# Autodesk Inventor assembly: 1_Body
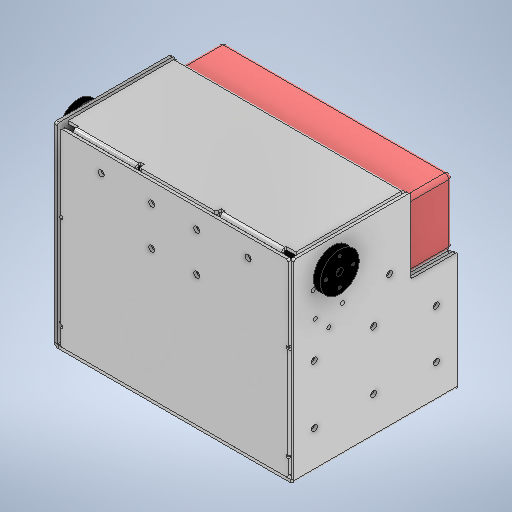
[picture p0: Inventor's stored thumbnail of the model, 512x512]
Saved by Autodesk Inventor 2025.2 (Build 292293000, 293)
## iProperties
Created: 2025-05-30
Part Number: 1_Body
Document SubType Name: Assembly
Designer: chris
Author: chris
## Documents named in this file (13)
- C:\Users\chris\Documents\Inventor\RHp_Humanoid_ver1\Assembly\1_Body.iam
- C:\Users\chris\Documents\Inventor\RHp_Humanoid_ver1\Part\Frame\Body\body_main_frame.ipt
- C:\Users\chris\Documents\Inventor\RHp_Humanoid_ver1\Part\Frame\Body\body_back_frame.ipt
- C:\Users\chris\Documents\Inventor\RHp_Humanoid_ver1\Part\Frame\Body\body_front_frame.ipt
- C:\Users\chris\Documents\Inventor\RHp_Humanoid_ver1\Part\Frame\Body\body_middle_frame.ipt
- C:\Users\chris\Documents\Inventor\RHp_Humanoid_ver1\Part\Frame\Body\body_motor_L_frame.ipt
- C:\Users\chris\Documents\Inventor\RHp_Humanoid_ver1\Part\Frame\Body\body_motor_R_frame.ipt
- C:\Users\chris\Documents\Inventor\RHp_Humanoid_ver1\Part\Frame\Body\body_top_frame.ipt
- C:\Users\chris\Documents\Inventor\RHp_Humanoid_ver1\Part\Other Parts\Servo_Driver.ipt
- C:\Users\chris\Documents\Inventor\RHp_Humanoid_ver1\Part\Other Parts\Battery_Pack.ipt
- C:\Users\chris\Documents\Inventor\RHp_Humanoid_ver1\Part\Other Parts\jetson_orin_super.ipt
- C:\Users\chris\Documents\Inventor\RHp_Humanoid_ver1\Part\HTD-45H, Horn\Horn\Top Horn.ipt
- C:\Users\chris\Documents\Inventor\RHp_Humanoid_ver1\Part\HTD-45H, Horn\HTD-45H\HTD-45H.iam
## Components (14 placed, 12 different names)
1. body_main_frame:1 — Mate:3, Flush:2, Mate:4, Mate:5, Flush:3, Flush:4, Mate:6, Flush:5, Mate:8, Mate:10, Mate:11, Flush:9, Flush:10, Mate:16, Mate:18, Flush:13, Mate:30, Flush:30, Flush:31, Mate:31, Mate:33
2. body_back_frame:1 — Mate:3, Flush:2, Mate:4, Mate:19
3. body_front_frame:1 — Mate:5, Flush:3, Flush:4, Flush:6, Mate:7, Flush:7, Mate:9, Flush:8
4. body_middle_frame:1 — Mate:6, Flush:5, Flush:6, Mate:17, Mate:28, Flush:29, Mate:29, Flush:32, Mate:32, Flush:33, Mate:34
5. body_motor_L_frame:1 — Mate:7, Flush:7, Mate:8
6. body_motor_R_frame:1 — Mate:9, Mate:10, Flush:8
7. body_top_frame:1 — Mate:11, Flush:9, Flush:10, Mate:20
8. Servo_Driver:1 — Mate:16, Mate:17, Mate:18
9. Battery_Pack:1 — Mate:19, Mate:20, Flush:13
10. jetson_orin_super:1 — Mate:28, Flush:29, Mate:29
11. Top Horn:1 — Rotational:1
12. Top Horn:2 — Rotational:2
13. HTD-45H:1 [sub-assembly] — Flush:32, Mate:31, Mate:32, Rotational:2
14. HTD-45H:2 [sub-assembly] — Flush:33, Mate:33, Mate:34, Rotational:1
## Relationships (38: Mate 21, Flush 15, RevoluteJoint 2)
- Mate:3: body_main_frame:1 ↔ body_back_frame:1
- Flush:2: body_main_frame:1 ↔ body_back_frame:1
- Mate:4: body_main_frame:1 ↔ body_back_frame:1
- Mate:5: body_main_frame:1 ↔ body_front_frame:1
- Flush:3 (1.5 mm): body_main_frame:1 ↔ body_front_frame:1
- Flush:4: body_main_frame:1 ↔ body_front_frame:1
- Mate:6: body_main_frame:1 ↔ body_middle_frame:1
- Flush:5 (1.5 mm): body_main_frame:1 ↔ body_middle_frame:1
- Flush:6 (-30 mm): body_front_frame:1 ↔ body_middle_frame:1
- Mate:7: body_front_frame:1 ↔ body_motor_L_frame:1
- Flush:7: body_front_frame:1 ↔ body_motor_L_frame:1
- Mate:8 (40 mm): body_main_frame:1 ↔ body_motor_L_frame:1
- Mate:9: body_front_frame:1 ↔ body_motor_R_frame:1
- Mate:10 (40 mm): body_main_frame:1 ↔ body_motor_R_frame:1
- Mate:11: body_main_frame:1 ↔ body_top_frame:1
- Flush:8: body_front_frame:1 ↔ body_motor_R_frame:1
- Flush:9: body_main_frame:1 ↔ body_top_frame:1
- Flush:10 (1.5 mm): body_main_frame:1 ↔ body_top_frame:1
- Mate:16: body_main_frame:1 ↔ Servo_Driver:1
- Mate:17: body_middle_frame:1 ↔ Servo_Driver:1
- Mate:18 (31 mm): body_main_frame:1 ↔ Servo_Driver:1
- Mate:19: body_back_frame:1 ↔ Battery_Pack:1
- Mate:20: body_top_frame:1 ↔ Battery_Pack:1
- Flush:13 (-2.5 mm): body_main_frame:1 ↔ Battery_Pack:1
- Mate:28: body_middle_frame:1 ↔ jetson_orin_super:1
- Flush:29 (6 mm): body_middle_frame:1 ↔ jetson_orin_super:1
- Mate:29 (7 mm): body_middle_frame:1 ↔ jetson_orin_super:1
- Mate:30: body_main_frame:1
- Flush:30: body_main_frame:1
- Flush:31: body_main_frame:1
- Flush:32: body_middle_frame:1 ↔ HTD-45H:1
- Mate:31: body_main_frame:1 ↔ HTD-45H:1
- Mate:32 (2 mm): body_middle_frame:1 ↔ HTD-45H:1
- Flush:33: body_middle_frame:1 ↔ HTD-45H:2
- Mate:33: body_main_frame:1 ↔ HTD-45H:2
- Mate:34 (2 mm): body_middle_frame:1 ↔ HTD-45H:2
- Rotational:1 [RevoluteJoint]: Top Horn:1 ↔ HTD-45H:2
- Rotational:2 [RevoluteJoint]: Top Horn:2 ↔ HTD-45H:1
